# Autodesk Inventor assembly: NOTGATEASSEMBLY
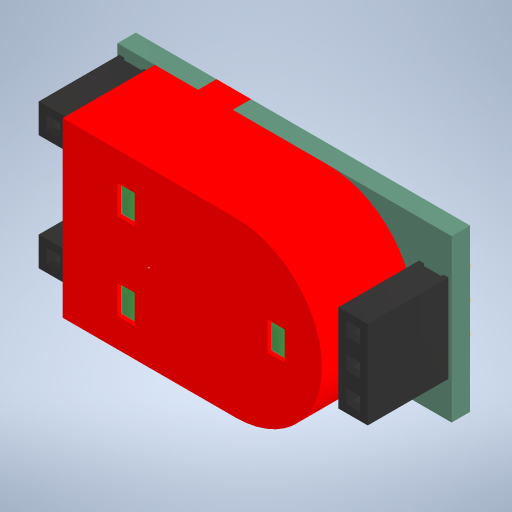
[picture p0: Inventor's stored thumbnail of the model, 512x512]
Saved by Autodesk Inventor 2024 (Build 280153000, 153)
## iProperties
Created: 2024-01-22
Part Number: NOTGATEASSEMBLY
Document SubType Name: Assembly
Designer: Jetsan
Author: Jetsan
## Documents named in this file (4)
- C:\Git\Personal\DigitalLogicProject\Models\NOTGATE\NOTGATEASSEMBLY.iam
- C:\Git\Personal\DigitalLogicProject\Models\ANDGATE\ANDGATE.iam
- C:\Git\Personal\DigitalLogicProject\Models\ANDGATE\ANDGATE.ipt
- C:\Git\Personal\DigitalLogicProject\Models\LIGHTPIPING\LightPipe.ipt
## Components (5 placed, 2 different names)
1. ANDGATE:1 [sub-assembly] — Mate:1, Mate:2, Mate:3, Mate:10, Mate:12
2. ANDGATE:2 — Mate:4, Mate:5, Mate:6, Mate:7, Mate:8, Mate:9, Mate:10, Mate:11, Mate:12
3. LightPipe:1 — Mate:1, Mate:4, Mate:5, Mate:6
4. LightPipe:2 — Mate:3, Mate:7, Mate:8
5. LightPipe:3 — Mate:2, Mate:9, Mate:11
## Relationships (12: Mate 12)
- Mate:1: ANDGATE:1 ↔ LightPipe:1
- Mate:2: ANDGATE:1 ↔ LightPipe:3
- Mate:3: ANDGATE:1 ↔ LightPipe:2
- Mate:4: ANDGATE:2 ↔ LightPipe:1
- Mate:5: ANDGATE:2 ↔ LightPipe:1
- Mate:6: ANDGATE:2 ↔ LightPipe:1
- Mate:7: ANDGATE:2 ↔ LightPipe:2
- Mate:8: ANDGATE:2 ↔ LightPipe:2
- Mate:9: ANDGATE:2 ↔ LightPipe:3
- Mate:10: ANDGATE:1 ↔ ANDGATE:2
- Mate:11: ANDGATE:2 ↔ LightPipe:3
- Mate:12: ANDGATE:1 ↔ ANDGATE:2
